# Autodesk Inventor assembly: TwoTalonPlate
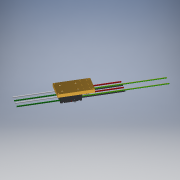
[picture p0: Inventor's stored thumbnail of the model, 180x180]
Saved by Autodesk Inventor 2019 (Build 230136000, 136)
## iProperties
Created: 2019-12-10
Part Number: TwoTalonPlate
Document SubType Name: Assembly
Designer: james
Author: james
## Documents named in this file (5)
- F:\JimsRobot\FIRSTRobots\Design\Library\Jims\TwoTalonPlate.iam
- F:\JimsRobot\FIRSTRobots\Design\Library\Jims\TalonSRXPlateTwo.ipt
- F:\JimsRobot\FIRSTRobots\Design\Library\CTR\Talon_SRX_14-838288\Talon_SRX_14-838288.ipt
- F:\JimsRobot\FIRSTRobots\Design\Library\CTR\CAN_CON_CAD\CAN_CON.ipt
- F:\JimsRobot\FIRSTRobots\Design\Library\McMaster\SocketScrews\91251A201_BLACK-OXIDE ALLOY STEEL SOCKET HEAD SCREW.ipt
## Components (10 placed, 4 different names)
1. TalonSRXPlateTwo:1 — Mate:1, Mate:2, Mate:3, Mate:4, Mate:5, Mate:6, Mate:7, Mate:8, Mate:9, Mate:10, Mate:11, Mate:12
2. Talon_SRX_14-838288:1 — Mate:4, Mate:5, Mate:6, Mate:13, Mate:14, Mate:19, Mate:20
3. Talon_SRX_14-838288:2 — Mate:1, Mate:2, Mate:3, Mate:15, Mate:16, Mate:17, Mate:18
4. CAN_CON:1 — Mate:8, Mate:11
5. CAN_CON:2 — Mate:7, Mate:12
6. CAN_CON:3 — Mate:9, Mate:10
7. 91251A201_BLACK-OXIDE ALLOY STEEL SOCKET HEAD SCREW:1 — Mate:13, Mate:20
8. 91251A201_BLACK-OXIDE ALLOY STEEL SOCKET HEAD SCREW:2 — Mate:14, Mate:19
9. 91251A201_BLACK-OXIDE ALLOY STEEL SOCKET HEAD SCREW:3 — Mate:15, Mate:18
10. 91251A201_BLACK-OXIDE ALLOY STEEL SOCKET HEAD SCREW:4 — Mate:16, Mate:17
## Relationships (20: Mate 20)
- Mate:1: TalonSRXPlateTwo:1 ↔ Talon_SRX_14-838288:2
- Mate:2: TalonSRXPlateTwo:1 ↔ Talon_SRX_14-838288:2
- Mate:3: TalonSRXPlateTwo:1 ↔ Talon_SRX_14-838288:2
- Mate:4: TalonSRXPlateTwo:1 ↔ Talon_SRX_14-838288:1
- Mate:5: TalonSRXPlateTwo:1 ↔ Talon_SRX_14-838288:1
- Mate:6: TalonSRXPlateTwo:1 ↔ Talon_SRX_14-838288:1
- Mate:7: TalonSRXPlateTwo:1 ↔ CAN_CON:2
- Mate:8: TalonSRXPlateTwo:1 ↔ CAN_CON:1
- Mate:9: TalonSRXPlateTwo:1 ↔ CAN_CON:3
- Mate:10: TalonSRXPlateTwo:1 ↔ CAN_CON:3
- Mate:11: TalonSRXPlateTwo:1 ↔ CAN_CON:1
- Mate:12: TalonSRXPlateTwo:1 ↔ CAN_CON:2
- Mate:13: Talon_SRX_14-838288:1 ↔ 91251A201_BLACK-OXIDE ALLOY STEEL SOCKET HEAD SCREW:1
- Mate:14: Talon_SRX_14-838288:1 ↔ 91251A201_BLACK-OXIDE ALLOY STEEL SOCKET HEAD SCREW:2
- Mate:15: Talon_SRX_14-838288:2 ↔ 91251A201_BLACK-OXIDE ALLOY STEEL SOCKET HEAD SCREW:3
- Mate:16: Talon_SRX_14-838288:2 ↔ 91251A201_BLACK-OXIDE ALLOY STEEL SOCKET HEAD SCREW:4
- Mate:17: Talon_SRX_14-838288:2 ↔ 91251A201_BLACK-OXIDE ALLOY STEEL SOCKET HEAD SCREW:4
- Mate:18: Talon_SRX_14-838288:2 ↔ 91251A201_BLACK-OXIDE ALLOY STEEL SOCKET HEAD SCREW:3
- Mate:19: Talon_SRX_14-838288:1 ↔ 91251A201_BLACK-OXIDE ALLOY STEEL SOCKET HEAD SCREW:2
- Mate:20: Talon_SRX_14-838288:1 ↔ 91251A201_BLACK-OXIDE ALLOY STEEL SOCKET HEAD SCREW:1
